# Autodesk Inventor assembly: FinalRev1
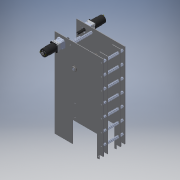
[picture p0: Inventor's stored thumbnail of the model, 180x180]
Saved by Autodesk Inventor 2016 (Build 200138000, 138)
## iProperties
Created: 2017-01-22
Part Number: FinalRev1
Document SubType Name: Assembly
Designer: madsenn
Author: madsenn
## Documents named in this file (12)
- C:\Users\Nick\Documents\GitHub\1073CAD\Robot2017\Assemblies\FinalRev1.iam
- C:\Users\Nick\Documents\GitHub\1073CAD\Robot2017\LauncherSidePlate.ipt
- C:\Users\Nick\Documents\GitHub\1073CAD\Robot2017\Parts\3InchChurro.ipt
- C:\Users\Nick\Documents\GitHub\1073CAD\Robot2017\GearboxPlateRev2.ipt
- C:\Users\Nick\Documents\GitHub\1073CAD\Robot2017\Parts\1InchChurro.ipt
- C:\Users\Nick\Documents\GitHub\1073CAD\Robot2017\VEXpro-CAD-Files-20170103\Motion\Gearboxes\VersaPlanetary Gearbox\VersaPlanetary v2\v2-VersaPlanetary-1stage-with-775pro-20161031.iam
- C:\Users\Nick\Documents\GitHub\1073CAD\Robot2017\VEXpro-CAD-Files-20170103\Motion\Bearings\217-3875-STEP-20140818.ipt
- C:\Users\Nick\Documents\GitHub\1073CAD\Robot2017\Parts\am-3480+4IN+Compliant+Wheel.ipt
- C:\Users\Nick\Documents\GitHub\1073CAD\Robot2017\Parts\FlywheelAxle.ipt
- C:\Users\Nick\Documents\GitHub\1073CAD\Robot2017\Parts\5,25InchChurro.ipt
- C:\Users\Nick\Documents\GitHub\1073CAD\Robot2017\Parts\HexShaftCollar.ipt
- C:\Users\Nick\Documents\GitHub\1073CAD\Robot2017\Parts\Spacer217-3261-STEP.ipt
## Components (46 placed, 11 different names)
1. LauncherSidePlate:1 — Mate:3, Mate:4, Mate:5, Mate:6, Mate:7, Mate:8, Mate:9, Mate:10, Mate:11, Mate:12, Mate:13, Mate:14, Mate:15, Mate:16, Mate:17, Mate:18, Mate:19, Mate:20, Mate:81, Mate:82, Mate:83, Mate:84, Mate:85, Mate:86
2. LauncherSidePlate:2 — Mate:1, Mate:2, Mate:23, Mate:24, Mate:25, Mate:26, Mate:27, Mate:28, Mate:30, Mate:31, Mate:50, Mate:51, Mate:52, Mate:53, Mate:54, Mate:55, Mate:56, Mate:57, Mate:58, Mate:59, Mate:60, Mate:61, Mate:62
3. 3InchChurro:1 — Mate:5, Mate:6, Mate:23
4. 3InchChurro:2 — Mate:7, Mate:8, Mate:24
5. 3InchChurro:4 — Mate:9, Mate:10, Mate:25
6. 3InchChurro:5 — Mate:11, Mate:12, Mate:26
7. 3InchChurro:6 — Mate:15, Mate:16, Mate:28
8. 3InchChurro:7 — Mate:13, Mate:14, Mate:27
9. 3InchChurro:8 — Mate:17, Mate:18, Mate:31
10. 3InchChurro:9 — Mate:19, Mate:20, Mate:30
11. 3InchChurro:10 — Mate:1, Mate:2, Mate:3, Mate:4
12. GearboxPlateRev2:1 — Mate:32, Mate:33, Mate:34, Mate:35, Mate:36, Mate:37, Mate:38, Mate:39, Mate:40, Mate:41, Mate:42, Mate:43, Mate:44, Mate:45, Mate:46, Mate:47, Mate:48, Mate:49, Mate:87, Mate:88, Mate:89, Mate:90, Insert:2, Mate:95, Mate:96, Mate:97, Mate:98, Flush:1
13. GearboxPlateRev2:2 — Mate:63, Mate:64, Mate:65, Mate:66, Mate:67, Mate:68, Mate:69, Mate:70, Mate:71, Mate:72, Mate:73, Mate:74, Mate:75, Mate:76, Mate:77, Mate:78, Mate:79, Mate:80, Mate:91, Mate:92, Mate:93, Mate:94, Insert:1, Mate:99, Mate:100, Mate:101, Mate:102, Mate:112
14. 1InchChurro:1 — Mate:32, Mate:42, Mate:58
15. 1InchChurro:2 — Mate:33, Mate:43, Mate:59
16. 1InchChurro:3 — Mate:34, Mate:45, Mate:51, Mate:60
17. 1InchChurro:4 — Mate:35, Mate:36, Mate:57, Mate:61, Mate:62
18. 1InchChurro:5 — Mate:37, Mate:49, Mate:56
19. 1InchChurro:6 — Mate:38, Mate:48, Mate:55
20. 1InchChurro:7 — Mate:39, Mate:47, Mate:54
21. 1InchChurro:8 — Mate:40, Mate:46, Mate:52, Mate:53
22. 1InchChurro:9 — Mate:41, Mate:44, Mate:50
23. 1InchChurro:10 — Mate:71, Mate:72, Mate:81, Mate:84
24. 1InchChurro:11 — Mate:70, Mate:73
25. 1InchChurro:12 — Mate:69, Mate:74
26. 1InchChurro:13 — Mate:68, Mate:80
27. 1InchChurro:14 — Mate:67, Mate:79, Mate:85, Mate:86
28. 1InchChurro:15 — Mate:66, Mate:75, Mate:83
29. 1InchChurro:16 — Mate:65, Mate:76
30. 1InchChurro:17 — Mate:64, Mate:77
31. 1InchChurro:18 — Mate:63, Mate:78, Mate:82
32. v2-VersaPlanetary-1stage-with-775pro-20161031:1 [sub-assembly] — Mate:87, Mate:88, Mate:89, Mate:90
33. v2-VersaPlanetary-1stage-with-775pro-20161031:2 [sub-assembly] — Mate:91, Mate:92, Mate:93, Mate:94
34. 217-3875-STEP-20140818:1 — Insert:2, Mate:103, Mate:104, Mate:122, Mate:123
35. 217-3875-STEP-20140818:2 — Insert:1, Mate:105, Mate:106, Mate:121, Mate:124
36. am-3480+4IN+Compliant+Wheel:1 — Mate:107, Mate:108, Mate:111, Mate:129
37. am-3480+4IN+Compliant+Wheel:2 — Mate:109, Mate:110, Mate:111, Mate:112, Mate:137
38. FlywheelAxle:1 — Mate:103, Mate:104, Flush:1, Mate:105, Mate:106, Mate:107, Mate:108, Mate:109, Mate:110, Mate:113, Mate:114, Mate:115, Mate:116, Mate:117, Mate:118, Mate:119, Mate:120, Mate:133, Mate:134, Mate:135, Mate:136
39. 5,25InchChurro:1 — Mate:96, Mate:98, Mate:101, Mate:102
40. 5,25InchChurro:2 — Mate:95, Mate:97, Mate:99, Mate:100
41. HexShaftCollar:1 — Mate:113, Mate:114, Mate:122
42. HexShaftCollar:2 — Mate:119, Mate:120, Mate:121
43. HexShaftCollar:3 — Mate:117, Mate:118, Mate:124
44. HexShaftCollar:4 — Mate:115, Mate:116, Mate:123
45. Spacer217-3261-STEP:1 — Mate:129, Mate:133, Mate:134
46. Spacer217-3261-STEP:2 — Mate:135, Mate:136, Mate:137
## Relationships (130: Mate 127, Insert 2, Flush 1)
- Mate:1: LauncherSidePlate:2 ↔ 3InchChurro:10
- Mate:2: LauncherSidePlate:2 ↔ 3InchChurro:10
- Mate:3: LauncherSidePlate:1 ↔ 3InchChurro:10
- Mate:4: LauncherSidePlate:1 ↔ 3InchChurro:10
- Mate:5: LauncherSidePlate:1 ↔ 3InchChurro:1
- Mate:6: LauncherSidePlate:1 ↔ 3InchChurro:1
- Mate:7: LauncherSidePlate:1 ↔ 3InchChurro:2
- Mate:8: LauncherSidePlate:1 ↔ 3InchChurro:2
- Mate:9: LauncherSidePlate:1 ↔ 3InchChurro:4
- Mate:10: LauncherSidePlate:1 ↔ 3InchChurro:4
- Mate:11: LauncherSidePlate:1 ↔ 3InchChurro:5
- Mate:12: LauncherSidePlate:1 ↔ 3InchChurro:5
- Mate:13: LauncherSidePlate:1 ↔ 3InchChurro:7
- Mate:14: LauncherSidePlate:1 ↔ 3InchChurro:7
- Mate:15: LauncherSidePlate:1 ↔ 3InchChurro:6
- Mate:16: LauncherSidePlate:1 ↔ 3InchChurro:6
- Mate:17: LauncherSidePlate:1 ↔ 3InchChurro:8
- Mate:18: LauncherSidePlate:1 ↔ 3InchChurro:8
- Mate:19: LauncherSidePlate:1 ↔ 3InchChurro:9
- Mate:20: LauncherSidePlate:1 ↔ 3InchChurro:9
- Mate:23: LauncherSidePlate:2 ↔ 3InchChurro:1
- Mate:24: LauncherSidePlate:2 ↔ 3InchChurro:2
- Mate:25: LauncherSidePlate:2 ↔ 3InchChurro:4
- Mate:26: LauncherSidePlate:2 ↔ 3InchChurro:5
- Mate:27: LauncherSidePlate:2 ↔ 3InchChurro:7
- Mate:28: LauncherSidePlate:2 ↔ 3InchChurro:6
- Mate:30: LauncherSidePlate:2 ↔ 3InchChurro:9
- Mate:31: LauncherSidePlate:2 ↔ 3InchChurro:8
- Mate:32: GearboxPlateRev2:1 ↔ 1InchChurro:1
- Mate:33: GearboxPlateRev2:1 ↔ 1InchChurro:2
- Mate:34: GearboxPlateRev2:1 ↔ 1InchChurro:3
- Mate:35: GearboxPlateRev2:1 ↔ 1InchChurro:4
- Mate:36: GearboxPlateRev2:1 ↔ 1InchChurro:4
- Mate:37: GearboxPlateRev2:1 ↔ 1InchChurro:5
- Mate:38: GearboxPlateRev2:1 ↔ 1InchChurro:6
- Mate:39: GearboxPlateRev2:1 ↔ 1InchChurro:7
- Mate:40: GearboxPlateRev2:1 ↔ 1InchChurro:8
- Mate:41: GearboxPlateRev2:1 ↔ 1InchChurro:9
- Mate:42: GearboxPlateRev2:1 ↔ 1InchChurro:1
- Mate:43: GearboxPlateRev2:1 ↔ 1InchChurro:2
- Mate:44: GearboxPlateRev2:1 ↔ 1InchChurro:9
- Mate:45: GearboxPlateRev2:1 ↔ 1InchChurro:3
- Mate:46: GearboxPlateRev2:1 ↔ 1InchChurro:8
- Mate:47: GearboxPlateRev2:1 ↔ 1InchChurro:7
- Mate:48: GearboxPlateRev2:1 ↔ 1InchChurro:6
- Mate:49: GearboxPlateRev2:1 ↔ 1InchChurro:5
- Mate:50: LauncherSidePlate:2 ↔ 1InchChurro:9
- Mate:51: LauncherSidePlate:2 ↔ 1InchChurro:3
- Mate:52: LauncherSidePlate:2 ↔ 1InchChurro:8
- Mate:53: LauncherSidePlate:2 ↔ 1InchChurro:8
- Mate:54: LauncherSidePlate:2 ↔ 1InchChurro:7
- Mate:55: LauncherSidePlate:2 ↔ 1InchChurro:6
- Mate:56: LauncherSidePlate:2 ↔ 1InchChurro:5
- Mate:57: LauncherSidePlate:2 ↔ 1InchChurro:4
- Mate:58: LauncherSidePlate:2 ↔ 1InchChurro:1
- Mate:59: LauncherSidePlate:2 ↔ 1InchChurro:2
- Mate:60: LauncherSidePlate:2 ↔ 1InchChurro:3
- Mate:61: LauncherSidePlate:2 ↔ 1InchChurro:4
- Mate:62: LauncherSidePlate:2 ↔ 1InchChurro:4
- Mate:63: GearboxPlateRev2:2 ↔ 1InchChurro:18
- Mate:64: GearboxPlateRev2:2 ↔ 1InchChurro:17
- Mate:65: GearboxPlateRev2:2 ↔ 1InchChurro:16
- Mate:66: GearboxPlateRev2:2 ↔ 1InchChurro:15
- Mate:67: GearboxPlateRev2:2 ↔ 1InchChurro:14
- Mate:68: GearboxPlateRev2:2 ↔ 1InchChurro:13
- Mate:69: GearboxPlateRev2:2 ↔ 1InchChurro:12
- Mate:70: GearboxPlateRev2:2 ↔ 1InchChurro:11
- Mate:71: GearboxPlateRev2:2 ↔ 1InchChurro:10
- Mate:72: GearboxPlateRev2:2 ↔ 1InchChurro:10
- Mate:73: GearboxPlateRev2:2 ↔ 1InchChurro:11
- Mate:74: GearboxPlateRev2:2 ↔ 1InchChurro:12
- Mate:75: GearboxPlateRev2:2 ↔ 1InchChurro:15
- Mate:76: GearboxPlateRev2:2 ↔ 1InchChurro:16
- Mate:77: GearboxPlateRev2:2 ↔ 1InchChurro:17
- Mate:78: GearboxPlateRev2:2 ↔ 1InchChurro:18
- Mate:79: GearboxPlateRev2:2 ↔ 1InchChurro:14
- Mate:80: GearboxPlateRev2:2 ↔ 1InchChurro:13
- Mate:81: LauncherSidePlate:1 ↔ 1InchChurro:10
- Mate:82: LauncherSidePlate:1 ↔ 1InchChurro:18
- Mate:83: LauncherSidePlate:1 ↔ 1InchChurro:15
- Mate:84: LauncherSidePlate:1 ↔ 1InchChurro:10
- Mate:85: LauncherSidePlate:1 ↔ 1InchChurro:14
- Mate:86: LauncherSidePlate:1 ↔ 1InchChurro:14
- Mate:87: GearboxPlateRev2:1 ↔ v2-VersaPlanetary-1stage-with-775pro-20161031:1
- Mate:88: GearboxPlateRev2:1 ↔ v2-VersaPlanetary-1stage-with-775pro-20161031:1
- Mate:89: GearboxPlateRev2:1 ↔ v2-VersaPlanetary-1stage-with-775pro-20161031:1
- Mate:90: GearboxPlateRev2:1 ↔ v2-VersaPlanetary-1stage-with-775pro-20161031:1
- Mate:91: GearboxPlateRev2:2 ↔ v2-VersaPlanetary-1stage-with-775pro-20161031:2
- Mate:92: GearboxPlateRev2:2 ↔ v2-VersaPlanetary-1stage-with-775pro-20161031:2
- Mate:93: GearboxPlateRev2:2 ↔ v2-VersaPlanetary-1stage-with-775pro-20161031:2
- Mate:94: GearboxPlateRev2:2 ↔ v2-VersaPlanetary-1stage-with-775pro-20161031:2
- Insert:1: GearboxPlateRev2:2 ↔ 217-3875-STEP-20140818:2
- Insert:2: GearboxPlateRev2:1 ↔ 217-3875-STEP-20140818:1
- Mate:95: GearboxPlateRev2:1 ↔ 5,25InchChurro:2
- Mate:96: GearboxPlateRev2:1 ↔ 5,25InchChurro:1
- Mate:97: GearboxPlateRev2:1 ↔ 5,25InchChurro:2
- Mate:98: GearboxPlateRev2:1 ↔ 5,25InchChurro:1
- Mate:99: GearboxPlateRev2:2 ↔ 5,25InchChurro:2
- Mate:100: GearboxPlateRev2:2 ↔ 5,25InchChurro:2
- Mate:101: GearboxPlateRev2:2 ↔ 5,25InchChurro:1
- Mate:102: GearboxPlateRev2:2 ↔ 5,25InchChurro:1
- Mate:103: 217-3875-STEP-20140818:1 ↔ FlywheelAxle:1
- Mate:104: 217-3875-STEP-20140818:1 ↔ FlywheelAxle:1
- Flush:1 (-7.9375 mm): GearboxPlateRev2:1 ↔ FlywheelAxle:1
- Mate:105: 217-3875-STEP-20140818:2 ↔ FlywheelAxle:1
- Mate:106: 217-3875-STEP-20140818:2 ↔ FlywheelAxle:1
- Mate:107: am-3480+4IN+Compliant+Wheel:1 ↔ FlywheelAxle:1
- Mate:108: am-3480+4IN+Compliant+Wheel:1 ↔ FlywheelAxle:1
- Mate:109: am-3480+4IN+Compliant+Wheel:2 ↔ FlywheelAxle:1
- Mate:110: am-3480+4IN+Compliant+Wheel:2 ↔ FlywheelAxle:1
- Mate:111: am-3480+4IN+Compliant+Wheel:1 ↔ am-3480+4IN+Compliant+Wheel:2
- Mate:112 (66.675 mm): GearboxPlateRev2:2 ↔ am-3480+4IN+Compliant+Wheel:2
- Mate:113: FlywheelAxle:1 ↔ HexShaftCollar:1
- Mate:114: FlywheelAxle:1 ↔ HexShaftCollar:1
- Mate:115: FlywheelAxle:1 ↔ HexShaftCollar:4
- Mate:116: FlywheelAxle:1 ↔ HexShaftCollar:4
- Mate:117: FlywheelAxle:1 ↔ HexShaftCollar:3
- Mate:118: FlywheelAxle:1 ↔ HexShaftCollar:3
- Mate:119: FlywheelAxle:1 ↔ HexShaftCollar:2
- Mate:120: FlywheelAxle:1 ↔ HexShaftCollar:2
- Mate:121: 217-3875-STEP-20140818:2 ↔ HexShaftCollar:2
- Mate:122: 217-3875-STEP-20140818:1 ↔ HexShaftCollar:1
- Mate:123: 217-3875-STEP-20140818:1 ↔ HexShaftCollar:4
- Mate:124: 217-3875-STEP-20140818:2 ↔ HexShaftCollar:3
- Mate:129: am-3480+4IN+Compliant+Wheel:1 ↔ Spacer217-3261-STEP:1
- Mate:133: FlywheelAxle:1 ↔ Spacer217-3261-STEP:1
- Mate:134: FlywheelAxle:1 ↔ Spacer217-3261-STEP:1
- Mate:135: FlywheelAxle:1 ↔ Spacer217-3261-STEP:2
- Mate:136: FlywheelAxle:1 ↔ Spacer217-3261-STEP:2
- Mate:137: am-3480+4IN+Compliant+Wheel:2 ↔ Spacer217-3261-STEP:2
